# Autodesk Inventor assembly: Innenhalter
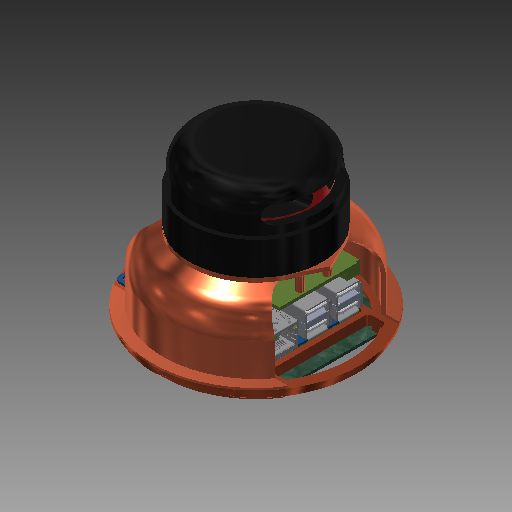
[picture p0: Inventor's stored thumbnail of the model, 512x512]
Saved by Autodesk Inventor 2018 (Build 220112000, 112)
## iProperties
Part Number: Innenhalter
Material: Generisch
Document SubType Name: Assembly
Designer: Jochen Alt
Mass: 252.875 g
Surface Area: 934.184 cm^2
Volume: 186.68 cm^3
Density: 1.35459 g/cm^3
Author: Jochen Alt
## Documents named in this file (8)
- D:\Projects\Manfred\cad\Inventor\Body Inside.iam
- D:\Projects\Manfred\cad\Inventor\ODroid C2\ODroid C2.iam
- D:\Projects\Manfred\cad\Inventor\ODroid Holder.ipt
- D:\Projects\Manfred\cad\Inventor\RPLidar A2.ipt
- D:\Projects\Manfred\cad\Inventor\Teensy 3.5-3.6.iam
- D:\Projects\Manfred\cad\Inventor\CortexPCB.ipt
- D:\Projects\Manfred\cad\Inventor\Lidar-Holder.ipt
- D:\Projects\Manfred\cad\Inventor\PCB Slamtec RPLidar A2.ipt
## Components (7 placed, 7 different names)
1. ODroid C2:1 [sub-assembly] — Passend:2, Passend:3, Passend:4
2. ODroid Holder:1 — Passend:1, Winkel:1, Passend:2, Passend:3, Passend:4, Passend:6, Winkel:4, Passend:8, Passend:14, Passend:15, Passend:16
3. RPLidar A2:1 — Passend:1, Winkel:1, Passend:7
4. Teensy 3.5/3.6:1 [sub-assembly] — Fluchtend:1
5. CortexPCB:1 — Passend:14, Passend:15, Passend:16, Fluchtend:1
6. Lidar-Holder:1 — Passend:6, Winkel:4, Passend:7, Passend:8, Passend:12, Passend:13
7. PCB Slamtec RPLidar A2:1 — Passend:12, Passend:13
## Relationships (15: Mate 12, Angle 2, Flush 1)
- Passend:1 [Mate]: ODroid Holder:1 ↔ RPLidar A2:1
- Winkel:1 [Angle] (144 deg): ODroid Holder:1 ↔ RPLidar A2:1
- Passend:2 [Mate]: ODroid C2:1 ↔ ODroid Holder:1
- Passend:3 [Mate]: ODroid C2:1 ↔ ODroid Holder:1
- Passend:4 [Mate]: ODroid C2:1 ↔ ODroid Holder:1
- Passend:6 [Mate]: ODroid Holder:1 ↔ Lidar-Holder:1
- Winkel:4 [Angle] (180 deg): ODroid Holder:1 ↔ Lidar-Holder:1
- Passend:7 [Mate]: RPLidar A2:1 ↔ Lidar-Holder:1
- Passend:8 [Mate]: ODroid Holder:1 ↔ Lidar-Holder:1
- Passend:12 [Mate]: Lidar-Holder:1 ↔ PCB Slamtec RPLidar A2:1
- Passend:13 [Mate]: Lidar-Holder:1 ↔ PCB Slamtec RPLidar A2:1
- Passend:14 [Mate]: ODroid Holder:1 ↔ CortexPCB:1
- Passend:15 [Mate]: ODroid Holder:1 ↔ CortexPCB:1
- Passend:16 [Mate]: ODroid Holder:1 ↔ CortexPCB:1
- Fluchtend:1 [Flush] (22 mm): Teensy 3.5/3.6:1 ↔ CortexPCB:1
